# Autodesk Inventor assembly: KWBH0001
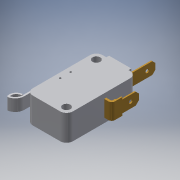
[picture p0: Inventor's stored thumbnail of the model, 180x180]
Saved by Autodesk Inventor 2016 (Build 200138000, 138)
## iProperties
Created: 2016-05-07
Part Number: KWBH0001
Document SubType Name: Assembly
Designer: agmle
Mass: 5.87832 g
Surface Area: 27.8836 cm^2
Volume: 4.57632 cm^3
Density: 1.28451 g/cm^3
Author: agmle
## Documents named in this file (6)
- C:\Users\agmle\BitTorrent Sync\private\projects\Creekfleet_Timer\hardware\CAD\Remote\Cherry_KWBH0001\KWBH0001.iam
- C:\Users\agmle\BitTorrent Sync\private\projects\Creekfleet_Timer\hardware\CAD\Remote\Cherry_KWBH0001\Housing.ipt
- C:\Users\agmle\BitTorrent Sync\private\projects\Creekfleet_Timer\hardware\CAD\Remote\Cherry_KWBH0001\Button.ipt
- C:\Users\agmle\BitTorrent Sync\private\projects\Creekfleet_Timer\hardware\CAD\Remote\Cherry_KWBH0001\NO_Contact.ipt
- C:\Users\agmle\BitTorrent Sync\private\projects\Creekfleet_Timer\hardware\CAD\Remote\Cherry_KWBH0001\COM_Contact.ipt
- C:\Users\agmle\BitTorrent Sync\private\projects\Creekfleet_Timer\hardware\CAD\Remote\Cherry_KWBH0001\Lever.ipt
## Components (5 placed, 5 different names)
1. Housing:1 — Mate:1, Mate:2, Mate:3, Mate:4, Mate:5, Mate:6, Mate:7, Mate:8, Mate:9, Tangent:1
2. Button:1 — Mate:1, Mate:2, Tangent:2
3. NO_Contact:1 — Mate:3, Mate:4, Mate:5
4. COM_Contact:1 — Mate:6, Mate:7, Mate:8
5. Lever:1 — Mate:9, Tangent:1, Tangent:2
## Relationships (11: Mate 9, Tangent 2)
- Mate:1: Housing:1 ↔ Button:1
- Mate:2 (0.25 mm): Housing:1 ↔ Button:1
- Mate:3: Housing:1 ↔ NO_Contact:1
- Mate:4: Housing:1 ↔ NO_Contact:1
- Mate:5: Housing:1 ↔ NO_Contact:1
- Mate:6: Housing:1 ↔ COM_Contact:1
- Mate:7: Housing:1 ↔ COM_Contact:1
- Mate:8: Housing:1 ↔ COM_Contact:1
- Mate:9: Housing:1 ↔ Lever:1
- Tangent:1: Housing:1 ↔ Lever:1
- Tangent:2: Button:1 ↔ Lever:1
